# Autodesk Inventor assembly: mini sand
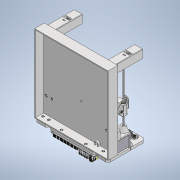
[picture p0: Inventor's stored thumbnail of the model, 180x180]
Saved by Autodesk Inventor 2022 (Build 260153000, 153)
## iProperties
Created: 2022-04-23
Part Number: mini sand
Document SubType Name: Assembly
Designer: Administrator
Title: mini sand v11
Author: Administrator
## Documents named in this file (29)
- Y:\Projects\Mini_Sand_Table\Mini Sand Table.iam
- Y:\Projects\Mini_Sand_Table\Hardware\Linear Rods\4mm x 140mm Rod.ipt
- Y:\Projects\Mini_Sand_Table\Hardware\Bearings\603ZZ Roller Bearing.ipt
- Y:\Projects\Mini_Sand_Table\Hardware\Linear Rods\4mm x 130mm Rod.ipt
- Y:\Projects\Mini_Sand_Table\Hardware\GT2 16T Pulley.ipt
- Y:\Projects\Mini_Sand_Table\Hardware\Magnet.ipt
- Y:\Projects\Mini_Sand_Table\Hardware\Bearings\LM4UU.ipt
- Y:\Projects\Mini_Sand_Table\3D Printed\Table Top.ipt
- Y:\Projects\Mini_Sand_Table\Electronics\NEMA 11.ipt
- Y:\Projects\Mini_Sand_Table\3D Printed\Belt Retainer.ipt
- Y:\Projects\Mini_Sand_Table\3D Printed\Magnet Mount Lower.ipt
- Y:\Projects\Mini_Sand_Table\3D Printed\Models with Heat Set Inserts\XY Joiner HSI.iam
- Y:\Projects\Mini_Sand_Table\3D Printed\Models with Heat Set Inserts\Idle Bearing Mount HSI.iam
- Y:\Projects\Mini_Sand_Table\Hardware\M3\Nuts\M3 Hex Nut.ipt
- Y:\Projects\Mini_Sand_Table\Hardware\4mm Ball.ipt
- Y:\Projects\Mini_Sand_Table\Electronics\SKR Mini E3 v3.0.ipt
- Y:\Projects\Mini_Sand_Table\3D Printed\Sand Cover.ipt
- Y:\Projects\Mini_Sand_Table\3D Printed\Models with Heat Set Inserts\Magnet Mount HSI.iam
- Y:\Projects\Mini_Sand_Table\3D Printed\Models with Heat Set Inserts\Motor Mount HSI.iam
- Y:\Projects\Mini_Sand_Table\3D Printed\Models with Heat Set Inserts\Driver Board Mount HSI.iam
- Y:\Projects\Mini_Sand_Table\Hardware\M2.5\M2.5 x 10 mm SHCS.ipt
- Y:\Projects\Mini_Sand_Table\Hardware\M2.5\M2.5 x 6 mm SHCS.ipt
- Y:\Projects\Mini_Sand_Table\Hardware\M3\Bolts\M3 x 16 mm FHCS.ipt
- Y:\Projects\Mini_Sand_Table\Hardware\M3\Bolts\M3 x 10 mm FHCS.ipt
- Y:\Projects\Mini_Sand_Table\Electronics\DC Jack.ipt
- Y:\Projects\Mini_Sand_Table\Electronics\DC Jack Nut.ipt
- Y:\Projects\Mini_Sand_Table\Hardware\M3\Nuts\5mm M3 Brass Standoff.ipt
- Y:\Projects\Mini_Sand_Table\Hardware\M3\Bolts\M3 x 25 mm FHCS.ipt
- Y:\Projects\Mini_Sand_Table\Hardware\M3\Bolts\M3 x 6 mm FHCS.ipt
## Components (90 placed, 30 different names)
1. M3 x 25 mm FHCS:1 — Insert:239
2. M3 x 25 mm FHCS:2 — Insert:238
3. M3 x 6 mm FHCS:1 — Insert:240
4. M3 x 6 mm FHCS:2 — Insert:243
5. M3 x 6 mm FHCS:3 — Insert:242
6. M3 x 6 mm FHCS:4 — Insert:241
7. M3 x 6 mm FHCS:5 — Insert:244
8. M3 x 6 mm FHCS:1 — Insert:245
9. M3 x 6 mm FHCS:2 — Insert:246
10. M3 x 6 mm FHCS:3 — Insert:249
11. M3 x 6 mm FHCS:4 — Insert:250
12. M3 x 6 mm FHCS:5 — Insert:247
13. M3 x 6 mm FHCS:6 — Insert:248
14. 5mm M3 Brass Standoff:5 — Insert:225
15. 5mm M3 Brass Standoff:4 — Insert:226
16. 5mm M3 Brass Standoff:3 — Insert:229
17. 5mm M3 Brass Standoff:2 — Insert:227
18. 5mm M3 Brass Standoff:1 — Insert:228
19. magnet:1 — Mate:31, Insert:107
20. 4mm x 140mm Rod:1 — Insert:60, Mate:46
21. 4mm x 140mm Rod:2 — Mate:9, Insert:61
22. 4mm x 130mm Rod:2 — Insert:95, Mate:43, Mate:45
23. 4mm x 130mm Rod:3 — Insert:87, Mate:44, Mate:49
24. GT2 16T Pulley:2 — Insert:68
25. gt2 pulley 16t v1:1 — Insert:65
26. 4mm Ball:1 — Mate:31, Tangent:1
27. Belt Retainer:2 — Insert:194, Insert:195
28. XY Joiner HSI:3 [sub-assembly] — Mate:44, Mate:45, Insert:202, Insert:232, Insert:233, Angle:1, Angle:2
29. Magnet Mount Lower:1 — Insert:159, Insert:196, Insert:197, Insert:230, Insert:231, Flush:3
30. Magnet Mount HSI:1 [sub-assembly] — Insert:107, Insert:230, Insert:231, Mate:50
31. Motor Mount HSI:1 [sub-assembly] — Insert:108, Insert:109, Insert:110, Insert:111, Insert:146, Insert:147
32. Motor Mount HSI:2 [sub-assembly] — Insert:112, Insert:113, Insert:114, Insert:148, Insert:149
33. table mount (1):1 [sub-assembly] — Insert:56, Insert:57, Insert:60, Insert:90, Insert:236, Angle:5, Insert:238
34. table mount (1):2 [sub-assembly] — Insert:58, Insert:59, Insert:61, Insert:89, Insert:237, Angle:6, Insert:239
35. XY Joiner HSI:2 [sub-assembly] — Insert:80, Insert:81, Insert:87, Insert:95, Insert:98, Insert:99, Insert:173, Insert:203, Insert:234, Insert:235, Angle:3, Angle:4
36. Belt Retainer:1 — Insert:82, Insert:83, Insert:198, Insert:199
37. Table Top:1 — Insert:56, Insert:57, Insert:58, Insert:59, Tangent:1, Mate:39, Mate:40, Mate:41, Insert:108, Insert:109, Insert:112, Insert:113, Insert:115, Insert:116, Insert:212, Insert:213, Insert:217, Insert:218, Insert:219, Insert:220, Insert:221, Insert:222, Insert:223, Insert:224, Insert:245, Insert:246, Insert:247, Insert:248, Insert:249, Insert:250
38. Driver Board Mount HSI:1 [sub-assembly] — Insert:115, Insert:116, Insert:142, Insert:143, Insert:144, Insert:145, Mate:47, Insert:200, Insert:201, Flush:1, Mate:48, Flush:2, Insert:225, Insert:226, Insert:227, Insert:228, Insert:229
39. Sand Cover:1 — Mate:39, Mate:40, Mate:41
40. DC Jack:1 — Insert:200
41. DC Jack Nut:1 — Insert:201
42. NEMA 11:1 — Insert:68, Insert:114, Mate:47
43. NEMA 11:2 — Insert:65, Insert:110, Insert:111
44. SKR Mini E3 v3.0:2 — Flush:1, Mate:48, Flush:2, Insert:240, Insert:241, Insert:242, Insert:243, Insert:244
45. LM4UU:3 — Mate:9, Insert:98
46. LM4UU:4 — Insert:99
47. LM4UU:5 — Insert:159, Mate:43
48. LM4UU:6 — Flush:3, Mate:49, Mate:50
49. LM4UU:7 — Mate:46
50. LM4UU:8
51. 603ZZ Roller Bearing:5 — Insert:81, Insert:82
52. 603ZZ Roller Bearing:6 — Insert:80, Insert:83
53. 603ZZ Roller Bearing:7
54. 603ZZ Roller Bearing:8
55. roller bearing:3 — Insert:90
56. roller bearing:4 — Insert:89
57. M3 Hex Nut:3 — Insert:236, Angle:5
58. M3 Hex Nut:4 — Insert:237, Angle:6
59. M3 Hex Nut:8 — Insert:232, Angle:2
60. M3 Hex Nut:7 — Insert:233, Angle:1
61. M3 Hex Nut:2 — Insert:234, Angle:4
62. M3 Hex Nut:6 — Insert:235, Angle:3
63. M3 x 10 mm FHCS:25 — Insert:222
64. M3 x 10 mm FHCS:24 — Insert:224
65. M3 x 10 mm FHCS:23 — Insert:223
66. M3 x 10 mm FHCS:7 — Insert:219
67. M3 x 10 mm FHCS:8 — Insert:212
68. M3 x 10 mm FHCS:9 — Insert:221
69. M3 x 10 mm FHCS:10 — Insert:213
70. M3 x 10 mm FHCS:11 — Insert:220
71. M3 x 10 mm FHCS:12 — Insert:217
72. M3 x 10 mm FHCS:15 — Insert:218
73. M3 x 10 mm FHCS:6 — Insert:199
74. M3 x 10 mm FHCS:5 — Insert:198
75. M3 x 10 mm FHCS:4 — Insert:197
76. M3 x 10 mm FHCS:3 — Insert:196
77. M3 x 10 mm FHCS:2 — Insert:195
78. M3 x 10 mm FHCS:1 — Insert:194
79. M3 x 16 mm FHCS:1 — Insert:173
80. M3 x 16 mm FHCS:2 — Insert:203
81. M3 x 16 mm FHCS:3
82. M3 x 16 mm FHCS:4 — Insert:202
83. M2.5 x 10 mm SHCS:1 — Insert:143
84. M2.5 x 10 mm SHCS:2 — Insert:142
85. M2.5 x 10 mm SHCS:3 — Insert:145
86. M2.5 x 10 mm SHCS:4 — Insert:144
87. M2.5 x 6 mm SHCS:1 — Insert:146
88. M2.5 x 6 mm SHCS:2 — Insert:147
89. M2.5 x 6 mm SHCS:3 — Insert:148
90. M2.5 x 6 mm SHCS:4 — Insert:149
## Relationships (114: Insert 91, Mate 13, Angle 6, Flush 3, Tangent 1)
- Mate:9: 4mm x 140mm Rod:2 ↔ LM4UU:3
- Insert:56: table mount (1):1 ↔ Table Top:1
- Insert:57: table mount (1):1 ↔ Table Top:1
- Insert:58: table mount (1):2 ↔ Table Top:1
- Insert:59: table mount (1):2 ↔ Table Top:1
- Insert:60: 4mm x 140mm Rod:1 ↔ table mount (1):1
- Insert:61: 4mm x 140mm Rod:2 ↔ table mount (1):2
- Insert:65: gt2 pulley 16t v1:1 ↔ NEMA 11:2
- Insert:68: GT2 16T Pulley:2 ↔ NEMA 11:1
- Insert:80: XY Joiner HSI:2 ↔ 603ZZ Roller Bearing:6
- Insert:81: XY Joiner HSI:2 ↔ 603ZZ Roller Bearing:5
- Insert:82: Belt Retainer:1 ↔ 603ZZ Roller Bearing:5
- Insert:83: Belt Retainer:1 ↔ 603ZZ Roller Bearing:6
- Insert:87: 4mm x 130mm Rod:3 ↔ XY Joiner HSI:2
- Insert:89: table mount (1):2 ↔ roller bearing:4
- Insert:90: table mount (1):1 ↔ roller bearing:3
- Insert:95: 4mm x 130mm Rod:2 ↔ XY Joiner HSI:2
- Insert:98: XY Joiner HSI:2 ↔ LM4UU:3
- Insert:99: XY Joiner HSI:2 ↔ LM4UU:4
- Mate:31: magnet:1 ↔ 4mm Ball:1
- Tangent:1: 4mm Ball:1 ↔ Table Top:1
- Mate:39: Table Top:1 ↔ Sand Cover:1
- Mate:40: Table Top:1 ↔ Sand Cover:1
- Mate:41: Table Top:1 ↔ Sand Cover:1
- Insert:107: magnet:1 ↔ Magnet Mount HSI:1
- Insert:108: Motor Mount HSI:1 ↔ Table Top:1
- Insert:109: Motor Mount HSI:1 ↔ Table Top:1
- Insert:110: Motor Mount HSI:1 ↔ NEMA 11:2
- Insert:111: Motor Mount HSI:1 ↔ NEMA 11:2
- Insert:112: Motor Mount HSI:2 ↔ Table Top:1
- Insert:113: Motor Mount HSI:2 ↔ Table Top:1
- Insert:114: Motor Mount HSI:2 ↔ NEMA 11:1
- Insert:115: Table Top:1 ↔ Driver Board Mount HSI:1
- Insert:116: Table Top:1 ↔ Driver Board Mount HSI:1
- Insert:142: Driver Board Mount HSI:1 ↔ M2.5 x 10 mm SHCS:2
- Insert:143: Driver Board Mount HSI:1 ↔ M2.5 x 10 mm SHCS:1
- Insert:144: Driver Board Mount HSI:1 ↔ M2.5 x 10 mm SHCS:4
- Insert:145: Driver Board Mount HSI:1 ↔ M2.5 x 10 mm SHCS:3
- Insert:146: Motor Mount HSI:1 ↔ M2.5 x 6 mm SHCS:1
- Insert:147: Motor Mount HSI:1 ↔ M2.5 x 6 mm SHCS:2
- Insert:148: Motor Mount HSI:2 ↔ M2.5 x 6 mm SHCS:3
- Insert:149: Motor Mount HSI:2 ↔ M2.5 x 6 mm SHCS:4
- Insert:159: Magnet Mount Lower:1 ↔ LM4UU:5
- Mate:43: 4mm x 130mm Rod:2 ↔ LM4UU:5
- Insert:173: XY Joiner HSI:2 ↔ M3 x 16 mm FHCS:1
- [Insert]: XY Joiner HSI:3 ↔ 603ZZ Roller Bearing:8
- [Insert]: XY Joiner HSI:3 ↔ 603ZZ Roller Bearing:7
- [Insert]: Belt Retainer:2 ↔ 603ZZ Roller Bearing:7
- [Insert]: Belt Retainer:2 ↔ 603ZZ Roller Bearing:8
- [Insert]: XY Joiner HSI:3 ↔ LM4UU:7
- [Insert]: XY Joiner HSI:3 ↔ LM4UU:8
- [Insert]: XY Joiner HSI:3 ↔ M3 x 16 mm FHCS:3
- Mate:44: 4mm x 130mm Rod:3 ↔ XY Joiner HSI:3
- Mate:45: 4mm x 130mm Rod:2 ↔ XY Joiner HSI:3
- Mate:46: 4mm x 140mm Rod:1 ↔ LM4UU:7
- Mate:47: Driver Board Mount HSI:1 ↔ NEMA 11:1
- Insert:194: Belt Retainer:2 ↔ M3 x 10 mm FHCS:1
- Insert:195: Belt Retainer:2 ↔ M3 x 10 mm FHCS:2
- Insert:196: Magnet Mount Lower:1 ↔ M3 x 10 mm FHCS:3
- Insert:197: Magnet Mount Lower:1 ↔ M3 x 10 mm FHCS:4
- Insert:198: Belt Retainer:1 ↔ M3 x 10 mm FHCS:5
- Insert:199: Belt Retainer:1 ↔ M3 x 10 mm FHCS:6
- Insert:200: Driver Board Mount HSI:1 ↔ DC Jack:1
- Insert:201: Driver Board Mount HSI:1 ↔ DC Jack Nut:1
- Insert:202: XY Joiner HSI:3 ↔ M3 x 16 mm FHCS:4
- Insert:203: XY Joiner HSI:2 ↔ M3 x 16 mm FHCS:2
- Insert:212: Table Top:1 ↔ M3 x 10 mm FHCS:8
- Insert:213: Table Top:1 ↔ M3 x 10 mm FHCS:10
- Insert:217: Table Top:1 ↔ M3 x 10 mm FHCS:12
- Insert:218: Table Top:1 ↔ M3 x 10 mm FHCS:15
- Insert:219: Table Top:1 ↔ M3 x 10 mm FHCS:7
- Insert:220: Table Top:1 ↔ M3 x 10 mm FHCS:11
- Insert:221: Table Top:1 ↔ M3 x 10 mm FHCS:9
- Flush:1 (2 mm): Driver Board Mount HSI:1 ↔ SKR Mini E3 v3.0:2
- Mate:48 (5 mm): Driver Board Mount HSI:1 ↔ SKR Mini E3 v3.0:2
- Flush:2 (3.35 mm): Driver Board Mount HSI:1 ↔ SKR Mini E3 v3.0:2
- Insert:222: Table Top:1 ↔ M3 x 10 mm FHCS:25
- Insert:223: Table Top:1 ↔ M3 x 10 mm FHCS:23
- Insert:224: Table Top:1 ↔ M3 x 10 mm FHCS:24
- Insert:225: 5mm M3 Brass Standoff:5 ↔ Driver Board Mount HSI:1
- Insert:226: 5mm M3 Brass Standoff:4 ↔ Driver Board Mount HSI:1
- Insert:227: 5mm M3 Brass Standoff:2 ↔ Driver Board Mount HSI:1
- Insert:228: 5mm M3 Brass Standoff:1 ↔ Driver Board Mount HSI:1
- Insert:229: 5mm M3 Brass Standoff:3 ↔ Driver Board Mount HSI:1
- Insert:230: Magnet Mount Lower:1 ↔ Magnet Mount HSI:1
- Insert:231: Magnet Mount Lower:1 ↔ Magnet Mount HSI:1
- Flush:3: Magnet Mount Lower:1 ↔ LM4UU:6
- Mate:49: 4mm x 130mm Rod:3 ↔ LM4UU:6
- Mate:50 (0.5 mm): Magnet Mount HSI:1 ↔ LM4UU:6
- Insert:232: XY Joiner HSI:3 ↔ M3 Hex Nut:8
- Insert:233: XY Joiner HSI:3 ↔ M3 Hex Nut:7
- Angle:1 (0 deg): XY Joiner HSI:3 ↔ M3 Hex Nut:7
- Angle:2 (0 deg): XY Joiner HSI:3 ↔ M3 Hex Nut:8
- Insert:234: XY Joiner HSI:2 ↔ M3 Hex Nut:2
- Insert:235: XY Joiner HSI:2 ↔ M3 Hex Nut:6
- Angle:3 (0 deg): XY Joiner HSI:2 ↔ M3 Hex Nut:6
- Angle:4 (0 deg): XY Joiner HSI:2 ↔ M3 Hex Nut:2
- Insert:236: table mount (1):1 ↔ M3 Hex Nut:3
- Angle:5 (0 deg): table mount (1):1 ↔ M3 Hex Nut:3
- Insert:237: table mount (1):2 ↔ M3 Hex Nut:4
- Angle:6 (0 deg): table mount (1):2 ↔ M3 Hex Nut:4
- Insert:238: M3 x 25 mm FHCS:2 ↔ table mount (1):1
- Insert:239: M3 x 25 mm FHCS:1 ↔ table mount (1):2
- Insert:240: M3 x 6 mm FHCS:1 ↔ SKR Mini E3 v3.0:2
- Insert:241: M3 x 6 mm FHCS:4 ↔ SKR Mini E3 v3.0:2
- Insert:242: M3 x 6 mm FHCS:3 ↔ SKR Mini E3 v3.0:2
- Insert:243: M3 x 6 mm FHCS:2 ↔ SKR Mini E3 v3.0:2
- Insert:244: M3 x 6 mm FHCS:5 ↔ SKR Mini E3 v3.0:2
- Insert:245: M3 x 6 mm FHCS:1 ↔ Table Top:1
- Insert:246: M3 x 6 mm FHCS:2 ↔ Table Top:1
- Insert:247: M3 x 6 mm FHCS:5 ↔ Table Top:1
- Insert:248: M3 x 6 mm FHCS:6 ↔ Table Top:1
- Insert:249: M3 x 6 mm FHCS:3 ↔ Table Top:1
- Insert:250: M3 x 6 mm FHCS:4 ↔ Table Top:1
## Named parameters: d265_d159 = 0 mm, d266_d160 = 0 mm, d267_d131 = 0 mm, d268_d132 = 0 mm, d269_d133 = 0 mm, d270_d134 = 0 mm, d275_d261 = 0 mm
